# Autodesk Inventor assembly: 000.012 - Крепление XT60 папа
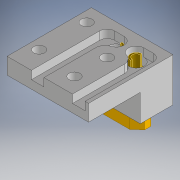
[picture p0: Inventor's stored thumbnail of the model, 180x180]
Saved by Autodesk Inventor 2022 (Build 260153000, 153)
## iProperties
Created: 2023-04-23
Part Number: 000.012 - Крепление XT60 папа
Document SubType Name: Assembly
Designer: Иван Петров
Author: Иван Петров
## Documents named in this file (3)
- C:\Users\Ivan Petrov\Documents\GitHub\OmniBot\design\000.012 - Крепление XT60 папа.iam
- C:\Users\Ivan Petrov\Documents\GitHub\OmniBot\design\000.012.001 - Основание.ipt
- C:\Users\Ivan Petrov\Documents\GitHub\OmniBot\design\standart_components\XT60FemaleConnector.ipt
## Components (2 placed, 2 different names)
1. 000.012.001 - Основание:1 — Совмещение:1
2. XT60FemaleConnector:1 — Совмещение:1
## Relationships (1: Mate 1)
- Совмещение:1 [Mate]: 000.012.001 - Основание:1 ↔ XT60FemaleConnector:1
